# Autodesk Inventor assembly: Cover Optical Camera Only
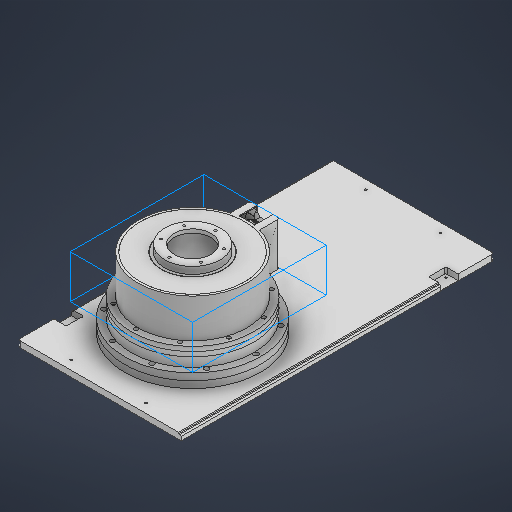
[picture p0: Inventor's stored thumbnail of the model, 512x512]
Saved by Autodesk Inventor 2025 (Build 290162000, 162)
## iProperties
Created: 2025-02-04
Part Number: Cover Optical Camera Only
Document SubType Name: Assembly
Designer: mayhe
Author: mayhe
## Documents named in this file (12)
- C:\Users\mayhe\OneDrive\Documents\GitHub\In-situ-monitoring-of-powder-bed-fusion-additive-manufacturing\system_development\Mithril\v0.2\Model\Cover Optical Camera Only.iam
- C:\Users\mayhe\OneDrive\Documents\GitHub\In-situ-monitoring-of-powder-bed-fusion-additive-manufacturing\system_development\Mithril\v0.2\Model\Cover (Optical Camera).ipt
- C:\Users\mayhe\OneDrive\Documents\GitHub\In-situ-monitoring-of-powder-bed-fusion-additive-manufacturing\system_development\Mithril\v0.2\Model\300mm Housing 1.ipt
- C:\Users\mayhe\OneDrive\Documents\GitHub\In-situ-monitoring-of-powder-bed-fusion-additive-manufacturing\system_development\Mithril\v0.2\Model\260 mm Glass.ipt
- C:\Users\mayhe\OneDrive\Documents\GitHub\In-situ-monitoring-of-powder-bed-fusion-additive-manufacturing\system_development\Mithril\v0.2\Model\Cylinder Spacer Optical Camera.ipt
- C:\Users\mayhe\OneDrive\Documents\GitHub\In-situ-monitoring-of-powder-bed-fusion-additive-manufacturing\system_development\Mithril\v0.2\Model\Cylinder Segment  Camera only.ipt
- C:\Users\mayhe\OneDrive\Documents\GitHub\In-situ-monitoring-of-powder-bed-fusion-additive-manufacturing\system_development\Mithril\v0.2\Model\Cylinder Slidey Bit Housing Camera only.ipt
- C:\Users\mayhe\OneDrive\Documents\GitHub\In-situ-monitoring-of-powder-bed-fusion-additive-manufacturing\system_development\Mithril\v0.2\Model\flircamera+lens.ipt
- C:\Users\mayhe\OneDrive\Documents\GitHub\In-situ-monitoring-of-powder-bed-fusion-additive-manufacturing\system_development\Mithril\v0.2\Model\300mm housing 2 Camera.ipt
- C:\Users\mayhe\OneDrive\Documents\GitHub\In-situ-monitoring-of-powder-bed-fusion-additive-manufacturing\system_development\Mithril\v0.2\Model\Cylinder Segment\Cylinder Segment Camera Only\C .Replace - Face.ipt
- C:\Users\mayhe\OneDrive\Documents\GitHub\In-situ-monitoring-of-powder-bed-fusion-additive-manufacturing\system_development\Mithril\v0.2\Model\Cylinder Segment\Cylinder Segment Camera Only.ipt
- C:\Users\mayhe\OneDrive\Documents\GitHub\In-situ-monitoring-of-powder-bed-fusion-additive-manufacturing\system_development\Mithril\v0.2\Model\Cylinder Segment\Cylinder Segment Camera Only\C .Replace - 10.ipt
## Components (10 placed, 10 different names)
1. Cover (Optical Camera):1 — Rotational:5
2. 300mm Housing 1:1 — Rotational:5, Rotational:11
3. 260 mm Glass:1
4. Cylinder Spacer Optical Camera:1 — Rotational:12, Mate:1
5. Cylinder Segment  Camera only:1 — Mate:1, Rotational:13, Cylindrical:1
6. Cylinder Slidey Bit Housing Camera only:1 — Rotational:13, Rotational:14
7. flircamera+lens:1 — Rotational:14
8. 300mm housing 2 Camera:2 — Rotational:11, Rotational:12
9. C .Replace - 10:2 — Cylindrical:1, Cylindrical:2
10. C .Replace - Face:3 — Cylindrical:2
## Relationships (8: RevoluteJoint 5, CylindricalJoint 2, Mate 1)
- Rotational:5 [RevoluteJoint]: Cover (Optical Camera):1 ↔ 300mm Housing 1:1
- Rotational:11 [RevoluteJoint]: 300mm Housing 1:1 ↔ 300mm housing 2 Camera:2
- Rotational:12 [RevoluteJoint]: Cylinder Spacer Optical Camera:1 ↔ 300mm housing 2 Camera:2
- Mate:1: Cylinder Spacer Optical Camera:1 ↔ Cylinder Segment  Camera only:1
- Rotational:13 [RevoluteJoint]: Cylinder Segment  Camera only:1 ↔ Cylinder Slidey Bit Housing Camera only:1
- Rotational:14 [RevoluteJoint]: Cylinder Slidey Bit Housing Camera only:1 ↔ flircamera+lens:1
- Cylindrical:1: Cylinder Segment  Camera only:1 ↔ C .Replace - 10:2
- Cylindrical:2: C .Replace - 10:2 ↔ C .Replace - Face:3
